# Autodesk Inventor assembly: Leg Module
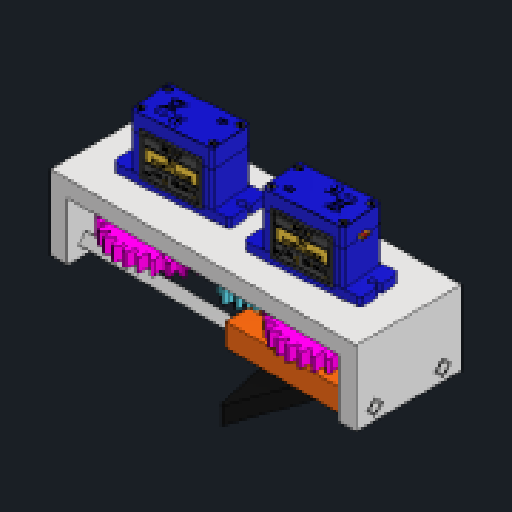
[picture p0: Inventor's stored thumbnail of the model, 512x512]
Saved by Autodesk Inventor 2023.2 (Build 272271030, 271C)
## iProperties
Created: 2024-02-28
Part Number: Leg Module
Document SubType Name: Assembly
Designer: robpl
Author: robpl
## Documents named in this file (8)
- C:\Users\robpl\OneDrive\Documents\Arduino\Onslaught\CAD\Onslaught V2\Leg Module.iam
- C:\Users\robpl\OneDrive\Documents\Arduino\Onslaught\CAD\Onslaught V2\Module Frame.ipt
- C:\Users\robpl\OneDrive\Documents\Arduino\Onslaught\CAD\SG90 - Micro Servo 9g - Tower Pro\SG90 - Micro Servo 9g - Tower Pro.ipt
- C:\Users\robpl\OneDrive\Documents\Arduino\Onslaught\CAD\Onslaught V2\Idler Gear.ipt
- C:\Users\robpl\OneDrive\Documents\Arduino\Onslaught\CAD\Onslaught V2\Leg.ipt
- C:\Users\robpl\OneDrive\Documents\Arduino\Onslaught\CAD\Onslaught V2\Rack.ipt
- C:\Users\robpl\OneDrive\Documents\Arduino\Onslaught\CAD\Onslaught V2\Servo Gear.ipt
- C:\Users\robpl\OneDrive\Documents\Arduino\Onslaught\CAD\Onslaught V2\Rail.ipt
## Components (12 placed, 7 different names)
1. Module Frame:1 — Mate:3, Mate:4, Mate:5, Mate:6, Mate:7, Mate:8, Mate:9, Mate:10, Mate:15, Mate:16, Mate:19, Angle:1, Flush:4, Mate:20, Angle:2, Flush:5
2. SG90 - Micro Servo 9g - Tower Pro:1 — Mate:3, Mate:4, Mate:5, Mate:12, Mate:13
3. SG90 - Micro Servo 9g - Tower Pro:2 — Mate:6, Mate:7, Mate:8, Mate:11, Mate:14
4. Idler Gear:1 — Mate:9, Flush:2, Flush:3
5. Leg:1 — Mate:17, Mate:18
6. Rack:1 — Mate:16, Flush:1, Flush:2, Mate:18
7. Servo Gear:1 — Mate:11, Mate:14
8. Idler Gear:2 — Mate:10, Flush:3
9. Rack:2 — Mate:15, Flush:1, Mate:17
10. Servo Gear:2 — Mate:12, Mate:13
11. Rail:1 — Mate:19, Angle:1, Flush:4
12. Rail:2 — Mate:20, Angle:2, Flush:5
## Relationships (25: Mate 18, Flush 5, Angle 2)
- Mate:3: Module Frame:1 ↔ SG90 - Micro Servo 9g - Tower Pro:1
- Mate:4: Module Frame:1 ↔ SG90 - Micro Servo 9g - Tower Pro:1
- Mate:5: Module Frame:1 ↔ SG90 - Micro Servo 9g - Tower Pro:1
- Mate:6: Module Frame:1 ↔ SG90 - Micro Servo 9g - Tower Pro:2
- Mate:7: Module Frame:1 ↔ SG90 - Micro Servo 9g - Tower Pro:2
- Mate:8: Module Frame:1 ↔ SG90 - Micro Servo 9g - Tower Pro:2
- Mate:9: Module Frame:1 ↔ Idler Gear:1
- Mate:10: Module Frame:1 ↔ Idler Gear:2
- Mate:11: SG90 - Micro Servo 9g - Tower Pro:2 ↔ Servo Gear:1
- Mate:12: SG90 - Micro Servo 9g - Tower Pro:1 ↔ Servo Gear:2
- Mate:13: SG90 - Micro Servo 9g - Tower Pro:1 ↔ Servo Gear:2
- Mate:14: SG90 - Micro Servo 9g - Tower Pro:2 ↔ Servo Gear:1
- Mate:15: Module Frame:1 ↔ Rack:2
- Mate:16: Module Frame:1 ↔ Rack:1
- Flush:1: Rack:1 ↔ Rack:2
- Mate:17 (-13.5 mm): Leg:1 ↔ Rack:2
- Flush:2 (-0.5 mm): Idler Gear:1 ↔ Rack:1
- Flush:3: Idler Gear:1 ↔ Idler Gear:2
- Mate:18 (1 mm): Leg:1 ↔ Rack:1
- Mate:19: Module Frame:1 ↔ Rail:1
- Angle:1 (0 deg): Module Frame:1 ↔ Rail:1
- Flush:4: Module Frame:1 ↔ Rail:1
- Mate:20: Module Frame:1 ↔ Rail:2
- Angle:2 (0 deg): Module Frame:1 ↔ Rail:2
- Flush:5: Module Frame:1 ↔ Rail:2
